# Autodesk Inventor assembly: Assembly1
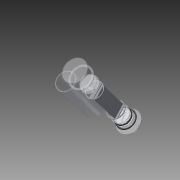
[picture p0: Inventor's stored thumbnail of the model, 180x180]
Saved by Autodesk Inventor 2015 (Build 190159000, 159)
## iProperties
Created: 2015-02-17
Part Number: Assembly1
Document SubType Name: Assembly
Designer: Hanjie
Author: Hanjie
## Documents named in this file (14)
- C:\Users\Hanjie\Desktop\2015Spring\vip\Assembly1.iam
- C:\Users\Hanjie\Desktop\2015Spring\vip\seal1.ipt
- C:\Users\Hanjie\Desktop\2015Spring\vip\seal2.ipt
- C:\Users\Hanjie\Desktop\2015Spring\vip\seal3.ipt
- C:\Users\Hanjie\Desktop\2015Spring\vip\tube.ipt
- C:\Users\Hanjie\Desktop\2015Spring\vip\open1.ipt
- C:\Users\Hanjie\Desktop\2015Spring\vip\open2.ipt
- C:\Users\Hanjie\Desktop\2015Spring\vip\open3.ipt
- C:\Users\Hanjie\Desktop\2015Spring\vip\open4.ipt
- C:\Users\Hanjie\Desktop\2015Spring\vip\open5.ipt
- C:\Users\Hanjie\Desktop\2015Spring\vip\oringlarge.ipt
- C:\Users\Hanjie\Desktop\2015Spring\vip\oringsmall.ipt
- C:\Users\Hanjie\Desktop\2015Spring\vip\baseboard.ipt
- C:\Users\Hanjie\Desktop\2015Spring\vip\fixpart.ipt
## Components (14 placed, 13 different names)
1. seal1:1 — Mate:2
2. seal2:1 — Mate:1, Mate:2
3. seal3:1 — Mate:1
4. tube:1
5. open1:1 — Mate:5, Mate:6
6. open2:1 — Mate:5, Mate:6, Mate:7
7. open3:1 — Mate:7, Mate:8, Mate:16
8. open4:1 — Mate:8, Mate:9
9. open5:1 — Mate:9, Mate:10
10. oringlarge:1 — Mate:10, Mate:11
11. oringsmall:1 — Mate:11
12. baseboard:1 — Mate:14, Mate:15
13. fixpart:1 — Mate:13, Mate:15, Mate:16
14. fixpart:2 — Mate:13, Mate:14
## Relationships (13: Mate 13)
- Mate:1: seal2:1 ↔ seal3:1
- Mate:2: seal1:1 ↔ seal2:1
- Mate:5: open1:1 ↔ open2:1
- Mate:6: open1:1 ↔ open2:1
- Mate:7: open2:1 ↔ open3:1
- Mate:8: open3:1 ↔ open4:1
- Mate:9: open4:1 ↔ open5:1
- Mate:10: open5:1 ↔ oringlarge:1
- Mate:11: oringlarge:1 ↔ oringsmall:1
- Mate:13: fixpart:1 ↔ fixpart:2
- Mate:14: baseboard:1 ↔ fixpart:2
- Mate:15: baseboard:1 ↔ fixpart:1
- Mate:16: open3:1 ↔ fixpart:1
